# Autodesk Inventor assembly: printer
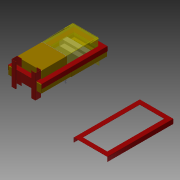
[picture p0: Inventor's stored thumbnail of the model, 180x180]
Saved by Autodesk Inventor 2014 SP2 (Build 180246200, 246)
## iProperties
Created: 2016-05-06
Part Number: printer
Document SubType Name: Assembly
Designer: cruiser
Author: cruiser
## Documents named in this file (10)
- C:\Users\cruiser\Desktop\models\3d printers\laserresin4\printer.iam
- C:\Users\cruiser\Desktop\models\3d printers\laserresin4\crane.ipt
- C:\Users\cruiser\Desktop\models\3d printers\laserresin4\carrier.ipt
- C:\Users\cruiser\Desktop\models\3d printers\laserresin4\reservoir.ipt
- C:\Users\cruiser\Desktop\models\3d printers\laserresin4\frame_inner.ipt
- C:\Users\cruiser\Desktop\models\3d printers\laserresin4\frame_lower.ipt
- C:\Users\cruiser\Desktop\models\3d printers\laserresin4\frame_face.ipt
- C:\Users\cruiser\Desktop\models\3d printers\laserresin4\door_assembly.iam
- C:\Users\cruiser\Desktop\models\3d printers\laserresin4\visor.ipt
- C:\Users\cruiser\Desktop\models\3d printers\laserresin4\frame_feet.ipt
## Components (11 placed, 9 different names)
1. crane:1 — Mate:1, Mate:2
2. carrier:1 — Mate:1, Mate:2, Mate:5, Mate:6, Mate:7, Mate:8, Mate:9, Mate:10, Mate:13
3. reservoir:1
4. frame_inner:1 — Mate:3, Flush:1, Mate:4, Flush:2, Mate:8, Mate:9, Mate:10, Mate:14, Mate:15
5. frame_lower:1 — Mate:5, Mate:6, Mate:7, Mate:11
6. frame_face:1
7. frame_face:2 — Mate:14, Mate:15
8. door_assembly:1 [sub-assembly] — Mate:12, Mate:13
9. visor:1 — Mate:3, Flush:1
10. visor:2 — Mate:4, Flush:2
11. frame_feet:1 — Mate:11, Mate:12
## Relationships (17: Mate 15, Flush 2)
- Mate:1: crane:1 ↔ carrier:1
- Mate:2: crane:1 ↔ carrier:1
- Mate:3: frame_inner:1 ↔ visor:1
- Flush:1: frame_inner:1 ↔ visor:1
- Mate:4: frame_inner:1 ↔ visor:2
- Flush:2: frame_inner:1 ↔ visor:2
- Mate:5: carrier:1 ↔ frame_lower:1
- Mate:6: carrier:1 ↔ frame_lower:1
- Mate:7: carrier:1 ↔ frame_lower:1
- Mate:8: carrier:1 ↔ frame_inner:1
- Mate:9: carrier:1 ↔ frame_inner:1
- Mate:10: carrier:1 ↔ frame_inner:1
- Mate:11: frame_lower:1 ↔ frame_feet:1
- Mate:12: door_assembly:1 ↔ frame_feet:1
- Mate:13: carrier:1 ↔ door_assembly:1
- Mate:14: frame_inner:1 ↔ frame_face:2
- Mate:15: frame_inner:1 ↔ frame_face:2
